# Autodesk Inventor assembly: NUCBase-PCB
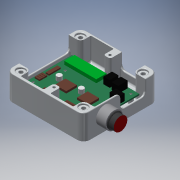
[picture p0: Inventor's stored thumbnail of the model, 180x180]
Saved by Autodesk Inventor 2016 (Build 200138000, 138)
## iProperties
Created: 2015-09-25
Part Number: NUCBase-PCB
Document SubType Name: Assembly
Designer: lachesis
Author: lachesis
## Documents named in this file (4)
- C:\Users\lachesis\git\Swarmie-Build\Swarmie-Assembly\Assemblies\NUCBase-PCB.iam
- C:\Users\lachesis\git\Swarmie-Build\Swarmie-Assembly\Parts\NUCBasePCB.ipt
- C:\Users\lachesis\git\Swarmie-Build\Swarmie-Assembly\Parts\PCB.ipt
- C:\Users\lachesis\git\Swarmie-Build\Swarmie-Assembly\Parts\SwitchPushButton.ipt
## Components (3 placed, 3 different names)
1. NUCBasePCB:1 — Rigid:1, Rigid:2
2. PCB:1 — Rigid:1
3. SwitchPushButton:1 — Rigid:2
## Relationships (2: WeldJoint 2)
- Rigid:1 [WeldJoint]: NUCBasePCB:1 ↔ PCB:1
- Rigid:2 [WeldJoint]: NUCBasePCB:1 ↔ SwitchPushButton:1
